# Autodesk Inventor assembly: Base Plate
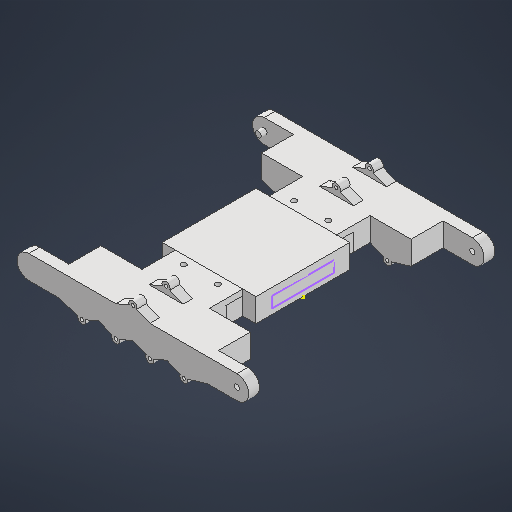
[picture p0: Inventor's stored thumbnail of the model, 512x512]
Saved by Autodesk Inventor 2026.2 (Build 302298010, 298A)
## iProperties
Created: 2026-07-10
Part Number: Base Plate
Document SubType Name: Assembly
Designer: icgre
Author: icgre
## Documents named in this file (4)
- C:\Users\Inigo Greenall\Documents\Excavator Project\Base Plate\Base Plate.iam
- C:\Users\Inigo Greenall\Documents\Excavator Project\Base Plate\Solid9.ipt
- C:\Users\Inigo Greenall\Documents\Excavator Project\Solid11.ipt
- C:\Users\Inigo Greenall\Documents\Excavator Project\Base Plate\Solid9_MIR.ipt
## Components (3 placed, 3 different names)
1. Solid9:1 — Mate:1, Angle:1, Flush:1, Flush:2
2. Solid11:1 — Mate:1, Angle:1, Flush:1, Flush:2, Mate:2, Angle:2, Flush:3, Flush:4
3. Solid9_MIR:1 — Mate:2, Angle:2, Flush:3, Flush:4
## Relationships (8: Flush 4, Mate 2, Angle 2)
- Mate:1: Solid9:1 ↔ Solid11:1
- Angle:1 (0 deg): Solid9:1 ↔ Solid11:1
- Flush:1: Solid9:1 ↔ Solid11:1
- Flush:2: Solid9:1 ↔ Solid11:1
- Mate:2: Solid11:1 ↔ Solid9_MIR:1
- Angle:2 (0 deg): Solid11:1 ↔ Solid9_MIR:1
- Flush:3: Solid11:1 ↔ Solid9_MIR:1
- Flush:4: Solid11:1 ↔ Solid9_MIR:1
